# Autodesk Inventor assembly: Y_Axis_LM3021
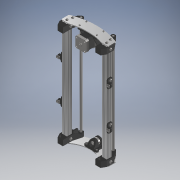
[picture p0: Inventor's stored thumbnail of the model, 180x180]
Saved by Autodesk Inventor 2020.2 (Build 242310000, 310)
## iProperties
Created: 2020-04-04
Part Number: Y_Axis_LM3021
Document SubType Name: Assembly
Designer: rah75
Author: rah75
## Documents named in this file (25)
- C:\Users\rah75\Documents\GitHub\LETU-Maker\CAD\Autodesk Inventor\Base_3001-5999\Y-Axis\Assemblies\Y_Axis_LM3021.iam
- C:\Users\rah75\Documents\GitHub\LETU-Maker\CAD\Autodesk Inventor\Base_3001-5999\Y-Axis\Printed_Parts\Y-Axis_Bearing_Mount_LM3012.ipt
- C:\Users\rah75\Documents\GitHub\LETU-Maker\CAD\Autodesk Inventor\Base_3001-5999\Y-Axis\Printed_Parts\Y-Axis_Foot_L_LM3014.ipt
- C:\Users\rah75\Documents\GitHub\LETU-Maker\CAD\Autodesk Inventor\Base_3001-5999\Y-Axis\Printed_Parts\Y-Axis_Motor_Mount_LM3017.ipt
- C:\Users\rah75\Documents\GitHub\LETU-Maker\CAD\Autodesk Inventor\Base_3001-5999\Y-Axis\Fabricated_Parts\Y-Axis_Motor_Plate_LM3018.ipt
- C:\Users\rah75\Documents\GitHub\LETU-Maker\CAD\Autodesk Inventor\Base_3001-5999\Y-Axis\Printed_Parts\Y-Axis_Foot_R_LM3016.ipt
- C:\Users\rah75\Documents\GitHub\LETU-Maker\CAD\Autodesk Inventor\Base_3001-5999\Y-Axis\Fabricated_Parts\Y-Axis_Extrusion_20x20x400mm_LM3020.ipt
- C:\Users\rah75\Documents\GitHub\LETU-Maker\CAD\Autodesk Inventor\Base_3001-5999\Y-Axis\Fabricated_Parts\Y-Axis_Bearing_Plate_LM3019.ipt
- C:\Users\rah75\Documents\GitHub\LETU-Maker\CAD\Autodesk Inventor\Base_3001-5999\Y-Axis\Printed_Parts\Y-Axis_Foot_w_Tap_R_LM3015.ipt
- C:\Users\rah75\Documents\GitHub\LETU-Maker\CAD\Autodesk Inventor\Stock_Components_1001-2999\Fasteners\Screws\BHHD_m5x10_LM1042.ipt
- C:\Users\rah75\Documents\GitHub\LETU-Maker\CAD\Autodesk Inventor\Stock_Components_1001-2999\Fasteners\Washers_Spacers\washer_m5_LM1002.ipt
- C:\Users\rah75\Documents\GitHub\LETU-Maker\CAD\Autodesk Inventor\Stock_Components_1001-2999\Fasteners\Nuts\heat_insert_m5_LM1018.ipt
- C:\Users\rah75\Documents\GitHub\LETU-Maker\CAD\Autodesk Inventor\Stock_Components_1001-2999\Fasteners\Nuts\heat_insert_m3_LM1017.ipt
- C:\Users\rah75\Documents\GitHub\LETU-Maker\CAD\Autodesk Inventor\Stock_Components_1001-2999\Fasteners\Nuts\hex_nut_m3_LM1019.ipt
- C:\Users\rah75\Documents\GitHub\LETU-Maker\CAD\Autodesk Inventor\Stock_Components_1001-2999\Fasteners\Screws\SHCS_m3x10_LM1015.ipt
- C:\Users\rah75\Documents\GitHub\LETU-Maker\CAD\Autodesk Inventor\Stock_Components_1001-2999\Motors\NEMA_17_LM1028.ipt
- C:\Users\rah75\Documents\GitHub\LETU-Maker\CAD\Autodesk Inventor\Stock_Components_1001-2999\Fasteners\Washers_Spacers\washer_m3_LM1001.ipt
- C:\Users\rah75\Documents\GitHub\LETU-Maker\CAD\Autodesk Inventor\Stock_Components_1001-2999\Power_Transmission\Bearings\608-ZZ_8x22mm_LM1028.ipt
- C:\Users\rah75\Documents\GitHub\LETU-Maker\CAD\Autodesk Inventor\Stock_Components_1001-2999\Fasteners\Nuts\hex_nut_m8_LM1043.ipt
- C:\Users\rah75\Documents\GitHub\LETU-Maker\CAD\Autodesk Inventor\Stock_Components_1001-2999\Fasteners\Screws\SHCS_m8x25_LM1044.ipt
- C:\Users\rah75\Documents\GitHub\LETU-Maker\CAD\Autodesk Inventor\Stock_Components_1001-2999\Structural\Linear_Motion_Shaft_8x400mm_LM1045.ipt
- C:\Users\rah75\Documents\GitHub\LETU-Maker\CAD\Autodesk Inventor\Stock_Components_1001-2999\Fasteners\Screws\Set Screws\set_screw_m3x6_LM1016.ipt
- C:\Users\rah75\Documents\GitHub\LETU-Maker\CAD\Autodesk Inventor\Stock_Components_1001-2999\Fasteners\Nuts\T_nut_m5_LM1021.ipt
- C:\Users\rah75\Documents\GitHub\LETU-Maker\CAD\Autodesk Inventor\Stock_Components_1001-2999\Power_Transmission\GT2_pulley_LM1034.ipt
- C:\Users\rah75\Documents\GitHub\LETU-Maker\CAD\Autodesk Inventor\Base_3001-5999\Y-Axis\Printed_Parts\Y-Axis_Extrusion_Bracket_LM3013.ipt
## Components (133 placed, 24 different names)
1. Y-Axis_Motor_Mount_LM3017:1 — Insert:1, Mate:1, Insert:54, Insert:55, Insert:56, Insert:57, Insert:66, Insert:71, Insert:72, Insert:73, Insert:74
2. Y-Axis_Motor_Plate_LM3018:1 — Insert:1, Mate:1, Insert:2, Insert:3, Insert:4, Insert:5, Insert:29, Insert:30, Insert:31, Insert:32, Insert:58, Insert:59, Insert:60, Insert:61
3. Y-Axis_Foot_L_LM3014:1 — Insert:2, Flush:1, Insert:35, Insert:41, Insert:44, Insert:47, Insert:78, Mate:9
4. Y-Axis_Foot_R_LM3016:1 — Insert:3, Flush:1, Insert:28, Insert:40, Insert:45, Insert:46, Insert:79
5. Y-Axis_Extrusion_20x20x400mm_LM3020:1 — Insert:5, Insert:6, Mate:4, Mate:7
6. Y-Axis_Extrusion_20x20x400mm_LM3020:2 — Insert:4, Mate:2, Mate:5, Mate:6
7. Y-Axis_Bearing_Plate_LM3019:1 — Insert:6, Mate:2, Insert:7, Insert:8, Insert:9, Mate:3, Insert:36, Insert:37, Insert:38, Insert:39, Insert:62, Insert:63, Insert:64, Insert:65
8. Y-Axis_Bearing_Mount_LM3012:1 — Insert:9, Mate:3, Insert:50, Insert:51, Insert:52, Insert:53, Insert:75, Insert:76, Insert:77
9. Y-Axis_Foot_L_LM3014:2 — Insert:8, Flush:2, Insert:27, Insert:34, Insert:43, Insert:48
10. Y-Axis_Foot_w_Tap_R_LM3015:1 — Insert:7, Flush:2, Insert:26, Insert:33, Insert:42, Insert:49
11. BHHD_m5x10_LM1042:1 — Insert:10
12. BHHD_m5x10_LM1042:2 — Insert:11
13. BHHD_m5x10_LM1042:3 — Insert:12
14. BHHD_m5x10_LM1042:4 — Insert:14
15. BHHD_m5x10_LM1042:5 — Insert:15
16. BHHD_m5x10_LM1042:6 — Insert:17
17. BHHD_m5x10_LM1042:7 — Insert:16
18. BHHD_m5x10_LM1042:8 — Insert:13
19. BHHD_m5x10_LM1042:9 — Insert:23
20. BHHD_m5x10_LM1042:10 — Insert:22
21. BHHD_m5x10_LM1042:11 — Insert:21
22. BHHD_m5x10_LM1042:12 — Insert:18
23. BHHD_m5x10_LM1042:13 — Insert:19
24. BHHD_m5x10_LM1042:14 — Insert:20
25. BHHD_m5x10_LM1042:15 — Insert:24
26. BHHD_m5x10_LM1042:16 — Insert:25
27. washer_m5_LM1002:1 — Insert:10, Insert:26, Insert:86
28. washer_m5_LM1002:2 — Insert:11, Insert:36
29. washer_m5_LM1002:3 — Insert:13, Insert:27, Insert:84
30. washer_m5_LM1002:4 — Insert:16, Insert:37
31. washer_m5_LM1002:5 — Insert:14, Insert:28, Insert:85
32. washer_m5_LM1002:6 — Insert:22, Insert:40, Insert:89
33. washer_m5_LM1002:7 — Insert:24, Insert:32
34. washer_m5_LM1002:8 — Insert:21, Insert:30
35. washer_m5_LM1002:9 — Insert:20, Insert:29
36. washer_m5_LM1002:10 — Insert:17, Insert:38
37. washer_m5_LM1002:11 — Insert:15, Insert:34, Insert:88
38. washer_m5_LM1002:12 — Insert:12, Insert:33, Insert:90
39. washer_m5_LM1002:13 — Insert:18, Insert:35, Insert:91
40. washer_m5_LM1002:14 — Insert:19, Insert:31
41. washer_m5_LM1002:15 — Insert:23, Insert:39
42. washer_m5_LM1002:16 — Insert:25, Insert:41, Insert:87
43. heat_insert_m5_LM1018:1 — Insert:44
44. heat_insert_m5_LM1018:2 — Insert:45
45. heat_insert_m5_LM1018:3 — Insert:43
46. heat_insert_m5_LM1018:4 — Insert:42
47. heat_insert_m3_LM1017:1 — Insert:49, Insert:82
48. heat_insert_m3_LM1017:2 — Insert:48, Insert:83
49. heat_insert_m3_LM1017:3 — Insert:47, Insert:81
50. heat_insert_m3_LM1017:4 — Insert:46, Insert:80
51. hex_nut_m3_LM1019:1 — Insert:56
52. hex_nut_m3_LM1019:2 — Insert:53
53. hex_nut_m3_LM1019:3 — Insert:52
54. hex_nut_m3_LM1019:4 — Insert:50
55. hex_nut_m3_LM1019:5 — Insert:51
56. hex_nut_m3_LM1019:6 — Insert:57
57. hex_nut_m3_LM1019:7 — Insert:55
58. hex_nut_m3_LM1019:8 — Insert:54
59. SHCS_m3x10_LM1015:1 — Insert:58
60. SHCS_m3x10_LM1015:2 — Insert:59
61. SHCS_m3x10_LM1015:3 — Insert:60
62. SHCS_m3x10_LM1015:4 — Insert:61
63. SHCS_m3x10_LM1015:5 — Insert:62
64. SHCS_m3x10_LM1015:6 — Insert:63
65. SHCS_m3x10_LM1015:7 — Insert:64
66. SHCS_m3x10_LM1015:8 — Insert:65
67. NEMA_17_LM1028:1 — Insert:66, Insert:92
68. SHCS_m3x10_LM1015:9 — Insert:70
69. SHCS_m3x10_LM1015:10 — Insert:69
70. SHCS_m3x10_LM1015:11 — Insert:68
71. SHCS_m3x10_LM1015:12 — Insert:67
72. washer_m3_LM1001:1 — Insert:67, Insert:74
73. washer_m3_LM1001:2 — Insert:68, Insert:73
74. washer_m3_LM1001:3 — Insert:69, Insert:71
75. washer_m3_LM1001:4 — Insert:70, Insert:72
76. 608-ZZ_8x22mm_LM1028:1 — Insert:75
77. hex_nut_m8_LM1043:1 — Insert:76
78. SHCS_m8x25_LM1044:1 — Insert:77
79. Linear_Motion_Shaft_8x400mm_LM1045:1 — Insert:79
80. Linear_Motion_Shaft_8x400mm_LM1045:2 — Insert:78
81. set_screw_m3x6_LM1016:1 — Insert:80
82. set_screw_m3x6_LM1016:2 — Insert:81
83. set_screw_m3x6_LM1016:3 — Insert:82
84. set_screw_m3x6_LM1016:4 — Insert:83
85. T_nut_m5_LM1021:1 — Insert:84
86. T_nut_m5_LM1021:2 — Insert:86
87. T_nut_m5_LM1021:3 — Insert:87
88. T_nut_m5_LM1021:4 — Insert:88
89. T_nut_m5_LM1021:5 — Insert:89
90. T_nut_m5_LM1021:6 — Insert:90
91. T_nut_m5_LM1021:7 — Insert:91, Flush:8
92. T_nut_m5_LM1021:8 — Insert:85, Flush:7
93. GT2_pulley_LM1034:1 — Insert:92
94. Y-Axis_Extrusion_Bracket_LM3013:1 — Mate:4, Flush:3, Flush:6, Insert:93, Insert:94, Insert:113, Insert:114, Insert:119
95. Y-Axis_Extrusion_Bracket_LM3013:2 — Mate:5, Flush:4, Flush:5, Insert:99, Insert:100, Mate:8, Insert:109, Insert:110, Insert:127
96. Y-Axis_Extrusion_Bracket_LM3013:3 — Mate:6, Flush:4, Flush:6, Insert:97, Insert:98, Mate:8, Mate:9, Insert:111, Insert:112, Insert:128
97. Y-Axis_Extrusion_Bracket_LM3013:4 — Mate:7, Flush:3, Flush:5, Insert:95, Insert:96, Insert:115, Insert:116, Insert:126
98. T_nut_m5_LM1021:9 — Insert:97
99. T_nut_m5_LM1021:10 — Insert:100
100. T_nut_m5_LM1021:11 — Insert:99
101. T_nut_m5_LM1021:12 — Insert:98, Flush:8
102. T_nut_m5_LM1021:13 — Insert:96
103. T_nut_m5_LM1021:14 — Insert:95
104. T_nut_m5_LM1021:15 — Insert:94
105. T_nut_m5_LM1021:16 — Insert:93, Flush:7
106. BHHD_m5x10_LM1042:17
107. washer_m5_LM1002:17 — Insert:113
108. BHHD_m5x10_LM1042:18
109. washer_m5_LM1002:18 — Insert:114
110. BHHD_m5x10_LM1042:19
111. washer_m5_LM1002:19 — Insert:115
112. BHHD_m5x10_LM1042:20
113. washer_m5_LM1002:20 — Insert:116
114. BHHD_m5x10_LM1042:21
115. washer_m5_LM1002:21 — Insert:112
116. BHHD_m5x10_LM1042:22
117. washer_m5_LM1002:22 — Insert:111
118. BHHD_m5x10_LM1042:23
119. washer_m5_LM1002:23 — Insert:109
120. BHHD_m5x10_LM1042:24
121. washer_m5_LM1002:24 — Insert:110
122. T_nut_m5_LM1021:17 — Insert:118, Flush:9
123. BHHD_m5x10_LM1042:25
124. washer_m5_LM1002:25 — Insert:118, Insert:119
125. T_nut_m5_LM1021:18 — Insert:121, Flush:9
126. BHHD_m5x10_LM1042:26
127. washer_m5_LM1002:26 — Insert:121, Insert:128
128. T_nut_m5_LM1021:19 — Insert:123, Flush:10
129. BHHD_m5x10_LM1042:27
130. washer_m5_LM1002:27 — Insert:123, Insert:127
131. T_nut_m5_LM1021:20 — Insert:125, Flush:10
132. BHHD_m5x10_LM1042:28
133. washer_m5_LM1002:28 — Insert:125, Insert:126
## Relationships (147: Insert 128, Flush 10, Mate 9)
- Insert:1: Y-Axis_Motor_Mount_LM3017:1 ↔ Y-Axis_Motor_Plate_LM3018:1
- Mate:1: Y-Axis_Motor_Mount_LM3017:1 ↔ Y-Axis_Motor_Plate_LM3018:1
- Insert:2: Y-Axis_Motor_Plate_LM3018:1 ↔ Y-Axis_Foot_L_LM3014:1
- Insert:3: Y-Axis_Motor_Plate_LM3018:1 ↔ Y-Axis_Foot_R_LM3016:1
- Flush:1: Y-Axis_Foot_L_LM3014:1 ↔ Y-Axis_Foot_R_LM3016:1
- Insert:4: Y-Axis_Motor_Plate_LM3018:1 ↔ Y-Axis_Extrusion_20x20x400mm_LM3020:2
- Insert:5: Y-Axis_Motor_Plate_LM3018:1 ↔ Y-Axis_Extrusion_20x20x400mm_LM3020:1
- Insert:6: Y-Axis_Extrusion_20x20x400mm_LM3020:1 ↔ Y-Axis_Bearing_Plate_LM3019:1
- Mate:2: Y-Axis_Extrusion_20x20x400mm_LM3020:2 ↔ Y-Axis_Bearing_Plate_LM3019:1
- Insert:7: Y-Axis_Bearing_Plate_LM3019:1 ↔ Y-Axis_Foot_w_Tap_R_LM3015:1
- Insert:8: Y-Axis_Bearing_Plate_LM3019:1 ↔ Y-Axis_Foot_L_LM3014:2
- Insert:9: Y-Axis_Bearing_Plate_LM3019:1 ↔ Y-Axis_Bearing_Mount_LM3012:1
- Flush:2: Y-Axis_Foot_L_LM3014:2 ↔ Y-Axis_Foot_w_Tap_R_LM3015:1
- Mate:3: Y-Axis_Bearing_Plate_LM3019:1 ↔ Y-Axis_Bearing_Mount_LM3012:1
- Insert:10: BHHD_m5x10_LM1042:1 ↔ washer_m5_LM1002:1
- Insert:11: BHHD_m5x10_LM1042:2 ↔ washer_m5_LM1002:2
- Insert:12: BHHD_m5x10_LM1042:3 ↔ washer_m5_LM1002:12
- Insert:13: BHHD_m5x10_LM1042:8 ↔ washer_m5_LM1002:3
- Insert:14: BHHD_m5x10_LM1042:4 ↔ washer_m5_LM1002:5
- Insert:15: BHHD_m5x10_LM1042:5 ↔ washer_m5_LM1002:11
- Insert:16: BHHD_m5x10_LM1042:7 ↔ washer_m5_LM1002:4
- Insert:17: BHHD_m5x10_LM1042:6 ↔ washer_m5_LM1002:10
- Insert:18: BHHD_m5x10_LM1042:12 ↔ washer_m5_LM1002:13
- Insert:19: BHHD_m5x10_LM1042:13 ↔ washer_m5_LM1002:14
- Insert:20: BHHD_m5x10_LM1042:14 ↔ washer_m5_LM1002:9
- Insert:21: BHHD_m5x10_LM1042:11 ↔ washer_m5_LM1002:8
- Insert:22: BHHD_m5x10_LM1042:10 ↔ washer_m5_LM1002:6
- Insert:23: BHHD_m5x10_LM1042:9 ↔ washer_m5_LM1002:15
- Insert:24: BHHD_m5x10_LM1042:15 ↔ washer_m5_LM1002:7
- Insert:25: BHHD_m5x10_LM1042:16 ↔ washer_m5_LM1002:16
- Insert:26: Y-Axis_Foot_w_Tap_R_LM3015:1 ↔ washer_m5_LM1002:1
- Insert:27: Y-Axis_Foot_L_LM3014:2 ↔ washer_m5_LM1002:3
- Insert:28: Y-Axis_Foot_R_LM3016:1 ↔ washer_m5_LM1002:5
- Insert:29: Y-Axis_Motor_Plate_LM3018:1 ↔ washer_m5_LM1002:9
- Insert:30: Y-Axis_Motor_Plate_LM3018:1 ↔ washer_m5_LM1002:8
- Insert:31: Y-Axis_Motor_Plate_LM3018:1 ↔ washer_m5_LM1002:14
- Insert:32: Y-Axis_Motor_Plate_LM3018:1 ↔ washer_m5_LM1002:7
- Insert:33: Y-Axis_Foot_w_Tap_R_LM3015:1 ↔ washer_m5_LM1002:12
- Insert:34: Y-Axis_Foot_L_LM3014:2 ↔ washer_m5_LM1002:11
- Insert:35: Y-Axis_Foot_L_LM3014:1 ↔ washer_m5_LM1002:13
- Insert:36: Y-Axis_Bearing_Plate_LM3019:1 ↔ washer_m5_LM1002:2
- Insert:37: Y-Axis_Bearing_Plate_LM3019:1 ↔ washer_m5_LM1002:4
- Insert:38: Y-Axis_Bearing_Plate_LM3019:1 ↔ washer_m5_LM1002:10
- Insert:39: Y-Axis_Bearing_Plate_LM3019:1 ↔ washer_m5_LM1002:15
- Insert:40: Y-Axis_Foot_R_LM3016:1 ↔ washer_m5_LM1002:6
- Insert:41: Y-Axis_Foot_L_LM3014:1 ↔ washer_m5_LM1002:16
- Insert:42: Y-Axis_Foot_w_Tap_R_LM3015:1 ↔ heat_insert_m5_LM1018:4
- Insert:43: Y-Axis_Foot_L_LM3014:2 ↔ heat_insert_m5_LM1018:3
- Insert:44: Y-Axis_Foot_L_LM3014:1 ↔ heat_insert_m5_LM1018:1
- Insert:45: Y-Axis_Foot_R_LM3016:1 ↔ heat_insert_m5_LM1018:2
- Insert:46: Y-Axis_Foot_R_LM3016:1 ↔ heat_insert_m3_LM1017:4
- Insert:47: Y-Axis_Foot_L_LM3014:1 ↔ heat_insert_m3_LM1017:3
- Insert:48: Y-Axis_Foot_L_LM3014:2 ↔ heat_insert_m3_LM1017:2
- Insert:49: Y-Axis_Foot_w_Tap_R_LM3015:1 ↔ heat_insert_m3_LM1017:1
- Insert:50: Y-Axis_Bearing_Mount_LM3012:1 ↔ hex_nut_m3_LM1019:4
- Insert:51: Y-Axis_Bearing_Mount_LM3012:1 ↔ hex_nut_m3_LM1019:5
- Insert:52: Y-Axis_Bearing_Mount_LM3012:1 ↔ hex_nut_m3_LM1019:3
- Insert:53: Y-Axis_Bearing_Mount_LM3012:1 ↔ hex_nut_m3_LM1019:2
- Insert:54: Y-Axis_Motor_Mount_LM3017:1 ↔ hex_nut_m3_LM1019:8
- Insert:55: Y-Axis_Motor_Mount_LM3017:1 ↔ hex_nut_m3_LM1019:7
- Insert:56: Y-Axis_Motor_Mount_LM3017:1 ↔ hex_nut_m3_LM1019:1
- Insert:57: Y-Axis_Motor_Mount_LM3017:1 ↔ hex_nut_m3_LM1019:6
- Insert:58: Y-Axis_Motor_Plate_LM3018:1 ↔ SHCS_m3x10_LM1015:1
- Insert:59: Y-Axis_Motor_Plate_LM3018:1 ↔ SHCS_m3x10_LM1015:2
- Insert:60: Y-Axis_Motor_Plate_LM3018:1 ↔ SHCS_m3x10_LM1015:3
- Insert:61: Y-Axis_Motor_Plate_LM3018:1 ↔ SHCS_m3x10_LM1015:4
- Insert:62: Y-Axis_Bearing_Plate_LM3019:1 ↔ SHCS_m3x10_LM1015:5
- Insert:63: Y-Axis_Bearing_Plate_LM3019:1 ↔ SHCS_m3x10_LM1015:6
- Insert:64: Y-Axis_Bearing_Plate_LM3019:1 ↔ SHCS_m3x10_LM1015:7
- Insert:65: Y-Axis_Bearing_Plate_LM3019:1 ↔ SHCS_m3x10_LM1015:8
- Insert:66: Y-Axis_Motor_Mount_LM3017:1 ↔ NEMA_17_LM1028:1
- Insert:67: SHCS_m3x10_LM1015:12 ↔ washer_m3_LM1001:1
- Insert:68: SHCS_m3x10_LM1015:11 ↔ washer_m3_LM1001:2
- Insert:69: SHCS_m3x10_LM1015:10 ↔ washer_m3_LM1001:3
- Insert:70: SHCS_m3x10_LM1015:9 ↔ washer_m3_LM1001:4
- Insert:71: Y-Axis_Motor_Mount_LM3017:1 ↔ washer_m3_LM1001:3
- Insert:72: Y-Axis_Motor_Mount_LM3017:1 ↔ washer_m3_LM1001:4
- Insert:73: Y-Axis_Motor_Mount_LM3017:1 ↔ washer_m3_LM1001:2
- Insert:74: Y-Axis_Motor_Mount_LM3017:1 ↔ washer_m3_LM1001:1
- Insert:75 (1 mm): Y-Axis_Bearing_Mount_LM3012:1 ↔ 608-ZZ_8x22mm_LM1028:1
- Insert:76: Y-Axis_Bearing_Mount_LM3012:1 ↔ hex_nut_m8_LM1043:1
- Insert:77: Y-Axis_Bearing_Mount_LM3012:1 ↔ SHCS_m8x25_LM1044:1
- Insert:78: Y-Axis_Foot_L_LM3014:1 ↔ Linear_Motion_Shaft_8x400mm_LM1045:2
- Insert:79: Y-Axis_Foot_R_LM3016:1 ↔ Linear_Motion_Shaft_8x400mm_LM1045:1
- Insert:80 (2 mm): heat_insert_m3_LM1017:4 ↔ set_screw_m3x6_LM1016:1
- Insert:81 (-2 mm): heat_insert_m3_LM1017:3 ↔ set_screw_m3x6_LM1016:2
- Insert:82 (-2 mm): heat_insert_m3_LM1017:1 ↔ set_screw_m3x6_LM1016:3
- Insert:83 (-2 mm): heat_insert_m3_LM1017:2 ↔ set_screw_m3x6_LM1016:4
- Insert:84 (6.375 mm): washer_m5_LM1002:3 ↔ T_nut_m5_LM1021:1
- Insert:85 (6.375 mm): washer_m5_LM1002:5 ↔ T_nut_m5_LM1021:8
- Insert:86 (6.375 mm): washer_m5_LM1002:1 ↔ T_nut_m5_LM1021:2
- Insert:87 (6.375 mm): washer_m5_LM1002:16 ↔ T_nut_m5_LM1021:3
- Insert:88 (6.375 mm): washer_m5_LM1002:11 ↔ T_nut_m5_LM1021:4
- Insert:89 (6.375 mm): washer_m5_LM1002:6 ↔ T_nut_m5_LM1021:5
- Insert:90 (6.375 mm): washer_m5_LM1002:12 ↔ T_nut_m5_LM1021:6
- Insert:91 (6.375 mm): washer_m5_LM1002:13 ↔ T_nut_m5_LM1021:7
- Insert:92: NEMA_17_LM1028:1 ↔ GT2_pulley_LM1034:1
- Mate:4: Y-Axis_Extrusion_20x20x400mm_LM3020:1 ↔ Y-Axis_Extrusion_Bracket_LM3013:1
- Mate:5: Y-Axis_Extrusion_20x20x400mm_LM3020:2 ↔ Y-Axis_Extrusion_Bracket_LM3013:2
- Mate:6: Y-Axis_Extrusion_20x20x400mm_LM3020:2 ↔ Y-Axis_Extrusion_Bracket_LM3013:3
- Mate:7: Y-Axis_Extrusion_20x20x400mm_LM3020:1 ↔ Y-Axis_Extrusion_Bracket_LM3013:4
- Flush:3: Y-Axis_Extrusion_Bracket_LM3013:1 ↔ Y-Axis_Extrusion_Bracket_LM3013:4
- Flush:4: Y-Axis_Extrusion_Bracket_LM3013:2 ↔ Y-Axis_Extrusion_Bracket_LM3013:3
- Flush:5: Y-Axis_Extrusion_Bracket_LM3013:2 ↔ Y-Axis_Extrusion_Bracket_LM3013:4
- Flush:6: Y-Axis_Extrusion_Bracket_LM3013:1 ↔ Y-Axis_Extrusion_Bracket_LM3013:3
- Insert:93 (6.375 mm): Y-Axis_Extrusion_Bracket_LM3013:1 ↔ T_nut_m5_LM1021:16
- Insert:94 (6.375 mm): Y-Axis_Extrusion_Bracket_LM3013:1 ↔ T_nut_m5_LM1021:15
- Insert:95 (6.375 mm): Y-Axis_Extrusion_Bracket_LM3013:4 ↔ T_nut_m5_LM1021:14
- Insert:96 (-6.375 mm): Y-Axis_Extrusion_Bracket_LM3013:4 ↔ T_nut_m5_LM1021:13
- Insert:97 (6.375 mm): Y-Axis_Extrusion_Bracket_LM3013:3 ↔ T_nut_m5_LM1021:9
- Insert:98 (-6.375 mm): Y-Axis_Extrusion_Bracket_LM3013:3 ↔ T_nut_m5_LM1021:12
- Insert:99 (6.375 mm): Y-Axis_Extrusion_Bracket_LM3013:2 ↔ T_nut_m5_LM1021:11
- Insert:100 (-6.375 mm): Y-Axis_Extrusion_Bracket_LM3013:2 ↔ T_nut_m5_LM1021:10
- Flush:7: T_nut_m5_LM1021:8 ↔ T_nut_m5_LM1021:16
- Flush:8: T_nut_m5_LM1021:7 ↔ T_nut_m5_LM1021:12
- Mate:8 (150 mm): Y-Axis_Extrusion_Bracket_LM3013:2 ↔ Y-Axis_Extrusion_Bracket_LM3013:3
- Mate:9 (-125 mm): Y-Axis_Foot_L_LM3014:1 ↔ Y-Axis_Extrusion_Bracket_LM3013:3
- [Insert]: BHHD_m5x10_LM1042:17 ↔ washer_m5_LM1002:17
- [Insert]: BHHD_m5x10_LM1042:18 ↔ washer_m5_LM1002:18
- [Insert]: BHHD_m5x10_LM1042:19 ↔ washer_m5_LM1002:19
- [Insert]: BHHD_m5x10_LM1042:20 ↔ washer_m5_LM1002:20
- [Insert]: BHHD_m5x10_LM1042:21 ↔ washer_m5_LM1002:21
- [Insert]: BHHD_m5x10_LM1042:22 ↔ washer_m5_LM1002:22
- [Insert]: BHHD_m5x10_LM1042:23 ↔ washer_m5_LM1002:23
- [Insert]: BHHD_m5x10_LM1042:24 ↔ washer_m5_LM1002:24
- Insert:109: Y-Axis_Extrusion_Bracket_LM3013:2 ↔ washer_m5_LM1002:23
- Insert:110: Y-Axis_Extrusion_Bracket_LM3013:2 ↔ washer_m5_LM1002:24
- Insert:111: Y-Axis_Extrusion_Bracket_LM3013:3 ↔ washer_m5_LM1002:22
- Insert:112: Y-Axis_Extrusion_Bracket_LM3013:3 ↔ washer_m5_LM1002:21
- Insert:113: Y-Axis_Extrusion_Bracket_LM3013:1 ↔ washer_m5_LM1002:17
- Insert:114: Y-Axis_Extrusion_Bracket_LM3013:1 ↔ washer_m5_LM1002:18
- Insert:115: Y-Axis_Extrusion_Bracket_LM3013:4 ↔ washer_m5_LM1002:19
- Insert:116: Y-Axis_Extrusion_Bracket_LM3013:4 ↔ washer_m5_LM1002:20
- [Insert]: BHHD_m5x10_LM1042:25 ↔ washer_m5_LM1002:25
- Insert:118 (6.375 mm): T_nut_m5_LM1021:17 ↔ washer_m5_LM1002:25
- Insert:119: Y-Axis_Extrusion_Bracket_LM3013:1 ↔ washer_m5_LM1002:25
- [Insert]: BHHD_m5x10_LM1042:26 ↔ washer_m5_LM1002:26
- Insert:121 (6.375 mm): T_nut_m5_LM1021:18 ↔ washer_m5_LM1002:26
- [Insert]: BHHD_m5x10_LM1042:27 ↔ washer_m5_LM1002:27
- Insert:123 (6.375 mm): T_nut_m5_LM1021:19 ↔ washer_m5_LM1002:27
- [Insert]: BHHD_m5x10_LM1042:28 ↔ washer_m5_LM1002:28
- Insert:125 (6.375 mm): T_nut_m5_LM1021:20 ↔ washer_m5_LM1002:28
- Insert:126: Y-Axis_Extrusion_Bracket_LM3013:4 ↔ washer_m5_LM1002:28
- Insert:127: Y-Axis_Extrusion_Bracket_LM3013:2 ↔ washer_m5_LM1002:27
- Insert:128: Y-Axis_Extrusion_Bracket_LM3013:3 ↔ washer_m5_LM1002:26
- Flush:9: T_nut_m5_LM1021:17 ↔ T_nut_m5_LM1021:18
- Flush:10: T_nut_m5_LM1021:19 ↔ T_nut_m5_LM1021:20
## Named parameters: d117_d22 = 0 mm, d118_d22 = 0 mm, d119_d22 = 0 mm, d120_d22 = 0 mm, d121_d22 = 0 mm, d122_d22 = 0 mm, d123_d22 = 0 mm, d124_d22 = 0 mm, d133_d118_d22 = 0 mm, d136_d133_d118_d22 = 0 mm, d137_d134 = 6.375 mm, d138_d133_d118_d22 = 0 mm, d139_d134 = 6.375 mm, d140_d133_d118_d22 = 0 mm, d141_d134 = 6.375 mm
